# Autodesk Inventor assembly: New
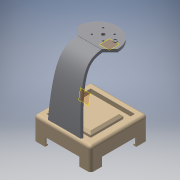
[picture p0: Inventor's stored thumbnail of the model, 180x180]
Saved by Autodesk Inventor 2016 (Build 200138000, 138)
## iProperties
Created: 2017-03-24
Part Number: New
Document SubType Name: Assembly
Designer: Jorian Bruslind
Author: Jorian Bruslind
## Documents named in this file (3)
- C:\Users\Jorian Bruslind\Documents\New.iam
- C:\Users\Jorian Bruslind\Desktop\Auto Terrarium\backplaterev2.0.ipt
- C:\Users\Jorian Bruslind\Desktop\Auto Terrarium\model for case.ipt
## Components (2 placed, 2 different names)
1. backplaterev2.0:1 — Mate:1, Mate:2
2. model for case:1 — Mate:1, Mate:2
## Relationships (2: Mate 2)
- Mate:1: backplaterev2.0:1 ↔ model for case:1
- Mate:2 (0.7937 mm): backplaterev2.0:1 ↔ model for case:1
